# Autodesk Inventor assembly: Sujecion centelladora
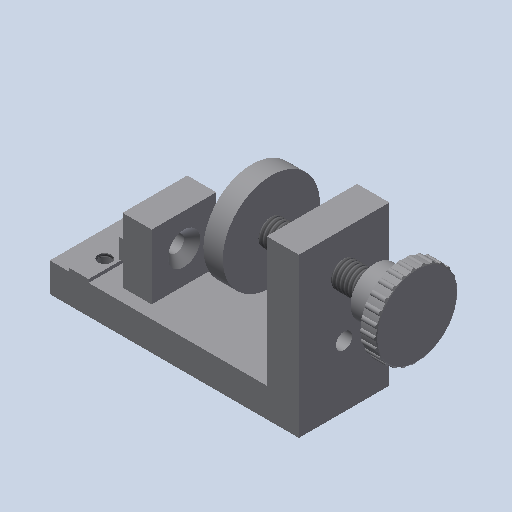
[picture p0: Inventor's stored thumbnail of the model, 512x512]
Saved by Autodesk Inventor 2024.2 (Build 282272000, 272)
## iProperties
Created: 2025-06-17
Part Number: Sujecion centelladora
Material: Genérico
Document SubType Name: Assembly
Designer: jd.castellanosq
Author: jd.castellanosq
## Documents named in this file (7)
- I:\MICROMECANICA\ALTAS ENERGIAS\Deteccion de Muones\Detectores centelladores\Partes Detector Centellador\SE Chasis DC\Partes Chasis DC\Sujecion centelladora.iam
- I:\MICROMECANICA\ALTAS ENERGIAS\Deteccion de Muones\Detectores centelladores\Partes Detector Centellador\SE Chasis DC\Partes Chasis DC\Base sujecion centelladora.ipt
- I:\MICROMECANICA\ALTAS ENERGIAS\Deteccion de Muones\Detectores centelladores\Partes Detector Centellador\SE Chasis DC\Partes Chasis DC\Guia sujecion centellador.ipt
- I:\MICROMECANICA\ALTAS ENERGIAS\Deteccion de Muones\Detectores centelladores\Partes Detector Centellador\SE Chasis DC\Partes Chasis DC\Tope guia.ipt
- I:\MICROMECANICA\ALTAS ENERGIAS\Deteccion de Muones\Detectores centelladores\Partes Detector Centellador\SE Chasis DC\Partes Chasis DC\Perilla.ipt
- I:\MICROMECANICA\ALTAS ENERGIAS\Deteccion de Muones\Detectores centelladores\Partes Detector Centellador\SE Chasis DC\Partes Chasis DC\mordaza.ipt
- I:\MICROMECANICA\ALTAS ENERGIAS\Deteccion de Muones\Detectores centelladores\Partes Detector Centellador\SE Chasis DC\Partes Chasis DC\Perilla sujecion.ipt
## Components (6 placed, 6 different names)
1. Base sujecion centelladora:1 — Mate:1, Mate:2, Flush:1, Mate:4, Mate:5, Mate:8, Mate:9, Mate:10, Mate:12
2. Guia sujecion centellador:1 — Mate:4, Mate:5, Mate:11, Mate:12
3. Tope guia:1 — Mate:8, Mate:9, Mate:10, Mate:17
4. Perilla:1 — Mate:11, Mate:13, Mate:14, Mate:18, Mate:19
5. mordaza:1 — Mate:13, Mate:14, Mate:17
6. Perilla sujecion:1 — Mate:18, Mate:19
## Relationships (15: Mate 14, Flush 1)
- Mate:1: Base sujecion centelladora:1
- Mate:2: Base sujecion centelladora:1
- Flush:1: Base sujecion centelladora:1
- Mate:4: Base sujecion centelladora:1 ↔ Guia sujecion centellador:1
- Mate:5: Base sujecion centelladora:1 ↔ Guia sujecion centellador:1
- Mate:8: Base sujecion centelladora:1 ↔ Tope guia:1
- Mate:9: Base sujecion centelladora:1 ↔ Tope guia:1
- Mate:10: Base sujecion centelladora:1 ↔ Tope guia:1
- Mate:11: Guia sujecion centellador:1 ↔ Perilla:1
- Mate:12: Base sujecion centelladora:1 ↔ Guia sujecion centellador:1
- Mate:13: Perilla:1 ↔ mordaza:1
- Mate:14: Perilla:1 ↔ mordaza:1
- Mate:17 (21 mm): Tope guia:1 ↔ mordaza:1
- Mate:18: Perilla:1 ↔ Perilla sujecion:1
- Mate:19: Perilla:1 ↔ Perilla sujecion:1
